# Autodesk Inventor assembly: demo gate
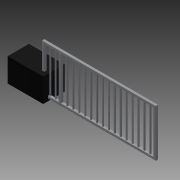
[picture p0: Inventor's stored thumbnail of the model, 180x180]
Saved by Autodesk Inventor 2019 (Build 230136000, 136)
## iProperties
Created: 2019-07-24
Part Number: demo gate
Document SubType Name: Assembly
Designer: brand
Author: brand
## Documents named in this file (3)
- C:\Users\Public\Documents\Autodesk\Inventor 2019\Templates\demo\demo gate.iam
- C:\Users\brand\Documents\GrabCAD\iLogic\demo\test demo.iam
- C:\Users\brand\Documents\GrabCAD\iLogic\demo\op demo.ipt
## Components (2 placed, 2 different names)
1. test demo:1 [sub-assembly] — Flush:1, Flush:2, Flush:3
2. op demo:1 — Flush:1, Flush:2, Flush:3
## Relationships (3: Flush 3)
- Flush:1 (-101.6 mm): test demo:1 ↔ op demo:1
- Flush:2 (-76.2 mm): test demo:1 ↔ op demo:1
- Flush:3 (50.8 mm): test demo:1 ↔ op demo:1
